# Autodesk Inventor assembly: Legassembly_MIR
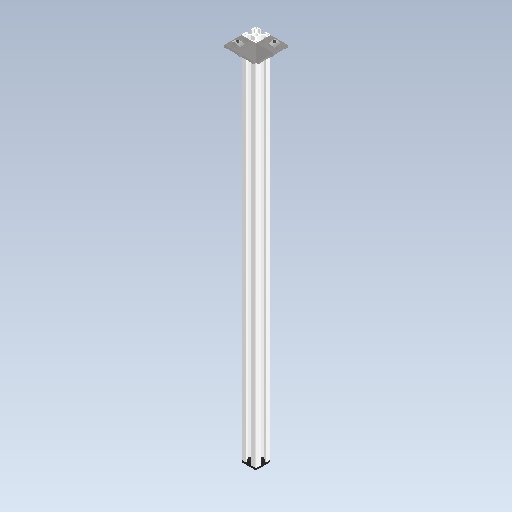
[picture p0: Inventor's stored thumbnail of the model, 512x512]
Saved by Autodesk Inventor 2020.2 (Build 242310000, 310)
## iProperties
Created: 2020-07-25
Part Number: Legassembly_MIR
Document SubType Name: Assembly
Designer: JK
Author: JK
## Documents named in this file (4)
- C:\Users\JK\Documents\Inventor\Mesa\Legassembly_MIR.iam
- C:\Users\JK\Documents\Inventor\Mesa\30x30x750_MIR.ipt
- C:\Users\JK\Documents\Inventor\Mesa\3030_endCap v4_MIR.ipt
- C:\Users\JK\Documents\Inventor\Mesa\Cornerassembly_MIR.iam
## Components (4 placed, 3 different names)
1. 30x30x750_MIR:1 — Flush:1, Flush:2, Mate:1, Flush:3, Mate:2, Flush:5, Flush:4, Mate:3
2. 3030_endCap v4_MIR:1 — Flush:1, Flush:2, Mate:1
3. Cornerassembly_MIR:1 [sub-assembly] — Flush:3, Mate:2
4. Cornerassembly_MIR:2 [sub-assembly] — Flush:5, Flush:4, Mate:3
## Relationships (8: Flush 5, Mate 3)
- Flush:1 (0.5 mm): 30x30x750_MIR:1 ↔ 3030_endCap v4_MIR:1
- Flush:2: 30x30x750_MIR:1 ↔ 3030_endCap v4_MIR:1
- Mate:1: 30x30x750_MIR:1 ↔ 3030_endCap v4_MIR:1
- Flush:3: 30x30x750_MIR:1 ↔ Cornerassembly_MIR:1
- Mate:2: 30x30x750_MIR:1 ↔ Cornerassembly_MIR:1
- Flush:5: 30x30x750_MIR:1 ↔ Cornerassembly_MIR:2
- Flush:4 (0.5 mm): 30x30x750_MIR:1 ↔ Cornerassembly_MIR:2
- Mate:3: 30x30x750_MIR:1 ↔ Cornerassembly_MIR:2
